# Autodesk Inventor assembly: 4x1inTractionWheel(Tire)-1111-2016_MIR
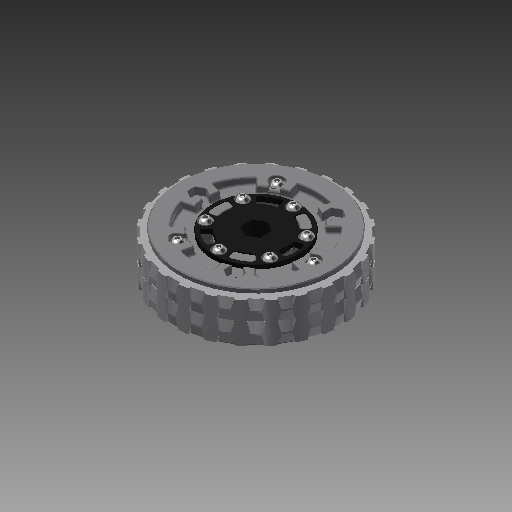
[picture p0: Inventor's stored thumbnail of the model, 512x512]
Saved by Autodesk Inventor 2018 (Build 220112000, 112)
## iProperties
Created: 2016-11-21
Part Number: 4x1inTractionWheel(Tire)-1111-2016_MIR
Document SubType Name: Assembly
Designer: Power Hawks CADD
Mass: 261.422 g
Surface Area: 1262.82 cm^2
Volume: 193.241 cm^3
Density: 1.35283 g/cm^3
Author: 589013
## Documents named in this file (9)
- F:\GrabCad\Resources\VEXpro Resources\Wheels\4 inch\4x1inTractionWheel(Tire)-1111-2016_MIR.iam
- F:\GrabCad\Resources\VEXpro Resources\Wheels\Wheel Parts\4InchWheelEnd-1111-2016_MIR.ipt
- F:\GrabCad\Resources\VEXpro Resources\Fasteners\Standoffs\Standoff0.75in-1111-2016_MIR.ipt
- F:\GrabCad\Resources\VEXpro Resources\Fasteners\Screws\Screw8-32x1.25in-1111-2016_MIR.ipt
- F:\GrabCad\Resources\VEXpro Resources\Fasteners\Nuts\Nut8-32Nylock-1111-2016_MIR.ipt
- F:\GrabCad\Resources\VEXpro Resources\Versa Motion\VersaHub(0.5inHex)-1111-2016_MIR.ipt
- F:\GrabCad\Resources\VEXpro Resources\Versa Motion\VersaHub(0.5inHex,Plastic)-1111-2016_MIR.ipt
- F:\GrabCad\Resources\VEXpro Resources\Fasteners\Screws\Screw8-32x0.5in-1111-2016_MIR.ipt
- F:\GrabCad\Resources\VEXpro Resources\Wheels\Wheel Parts\4InchTire\4inchTire-1111-2017_MIR.iam
## Components (30 placed, 8 different names)
1. 4InchWheelEnd-1111-2016_MIR:1 — Angle:1, Angle:2, Angle:4, Angle:3, Rotational:1, Rotational:3, Rotational:2, Rotational:6, Rotational:5, Rotational:4, Rotational:10, Rotational:9, Rigid:1
2. 4InchWheelEnd-1111-2016_MIR:2 — Insert:1, Insert:2, Insert:3, Rotational:3, Rotational:2, Rotational:8, Rotational:7, Rigid:2
3. Screw8-32x1.25in-1111-2016_MIR:1 — Insert:1
4. Screw8-32x1.25in-1111-2016_MIR:2 — Insert:2
5. Screw8-32x1.25in-1111-2016_MIR:3 — Insert:3
6. Nut8-32Nylock-1111-2016_MIR:1 — Angle:2, Rotational:6
7. Nut8-32Nylock-1111-2016_MIR:2 — Angle:4, Rotational:5
8. Nut8-32Nylock-1111-2016_MIR:3 — Angle:3, Rotational:4
9. VersaHub(0.5inHex)-1111-2016_MIR:1 — Insert:4, Insert:6, Insert:5, Insert:7, Insert:8, Insert:9, Rotational:8, Rotational:7
10. VersaHub(0.5inHex,Plastic)-1111-2016_MIR:1 — Insert:10, Insert:11, Insert:13, Insert:14, Insert:12, Insert:15, Rotational:10, Rotational:9
11. Screw8-32x0.5in-1111-2016_MIR:1 — Insert:4
12. Screw8-32x0.5in-1111-2016_MIR:2 — Insert:6
13. Screw8-32x0.5in-1111-2016_MIR:3 — Insert:5
14. Screw8-32x0.5in-1111-2016_MIR:4 — Insert:7
15. Screw8-32x0.5in-1111-2016_MIR:5 — Insert:8
16. Screw8-32x0.5in-1111-2016_MIR:6 — Insert:9
17. Screw8-32x0.5in-1111-2016_MIR:7 — Insert:10
18. Screw8-32x0.5in-1111-2016_MIR:8 — Insert:11
19. Screw8-32x0.5in-1111-2016_MIR:9 — Insert:13
20. Screw8-32x0.5in-1111-2016_MIR:10 — Insert:14
21. Screw8-32x0.5in-1111-2016_MIR:11 — Insert:12
22. Screw8-32x0.5in-1111-2016_MIR:12 — Insert:15
23. 4inchTire-1111-2017_MIR:1 [sub-assembly] — Rigid:1
24. 4inchTire-1111-2017_MIR:2 [sub-assembly] — Rigid:2
25. Standoff0.75in-1111-2016_MIR:1 — Angle:1, Rotational:1
26. Standoff0.75in-1111-2016_MIR:2
27. Standoff0.75in-1111-2016_MIR:3
28. Standoff0.75in-1111-2016_MIR:4
29. Standoff0.75in-1111-2016_MIR:5
30. Standoff0.75in-1111-2016_MIR:6
## Component patterns: (6 elements, first: Standoff0.75in-1111-2016_MIR:1)
## Relationships (31: Insert 15, RevoluteJoint 10, Angle 4, WeldJoint 2)
- Angle:1 (0 deg): 4InchWheelEnd-1111-2016_MIR:1 ↔ Standoff0.75in-1111-2016_MIR:1
- Insert:1: 4InchWheelEnd-1111-2016_MIR:2 ↔ Screw8-32x1.25in-1111-2016_MIR:1
- Insert:2: 4InchWheelEnd-1111-2016_MIR:2 ↔ Screw8-32x1.25in-1111-2016_MIR:2
- Insert:3: 4InchWheelEnd-1111-2016_MIR:2 ↔ Screw8-32x1.25in-1111-2016_MIR:3
- Angle:2 (0 deg): 4InchWheelEnd-1111-2016_MIR:1 ↔ Nut8-32Nylock-1111-2016_MIR:1
- Angle:4 (0 deg): 4InchWheelEnd-1111-2016_MIR:1 ↔ Nut8-32Nylock-1111-2016_MIR:2
- Angle:3 (0 deg): 4InchWheelEnd-1111-2016_MIR:1 ↔ Nut8-32Nylock-1111-2016_MIR:3
- Insert:4: VersaHub(0.5inHex)-1111-2016_MIR:1 ↔ Screw8-32x0.5in-1111-2016_MIR:1
- Insert:6: VersaHub(0.5inHex)-1111-2016_MIR:1 ↔ Screw8-32x0.5in-1111-2016_MIR:2
- Insert:5: VersaHub(0.5inHex)-1111-2016_MIR:1 ↔ Screw8-32x0.5in-1111-2016_MIR:3
- Insert:7: VersaHub(0.5inHex)-1111-2016_MIR:1 ↔ Screw8-32x0.5in-1111-2016_MIR:4
- Insert:8: VersaHub(0.5inHex)-1111-2016_MIR:1 ↔ Screw8-32x0.5in-1111-2016_MIR:5
- Insert:9: VersaHub(0.5inHex)-1111-2016_MIR:1 ↔ Screw8-32x0.5in-1111-2016_MIR:6
- Insert:10: VersaHub(0.5inHex,Plastic)-1111-2016_MIR:1 ↔ Screw8-32x0.5in-1111-2016_MIR:7
- Insert:11: VersaHub(0.5inHex,Plastic)-1111-2016_MIR:1 ↔ Screw8-32x0.5in-1111-2016_MIR:8
- Insert:13: VersaHub(0.5inHex,Plastic)-1111-2016_MIR:1 ↔ Screw8-32x0.5in-1111-2016_MIR:9
- Insert:14: VersaHub(0.5inHex,Plastic)-1111-2016_MIR:1 ↔ Screw8-32x0.5in-1111-2016_MIR:10
- Insert:12: VersaHub(0.5inHex,Plastic)-1111-2016_MIR:1 ↔ Screw8-32x0.5in-1111-2016_MIR:11
- Insert:15: VersaHub(0.5inHex,Plastic)-1111-2016_MIR:1 ↔ Screw8-32x0.5in-1111-2016_MIR:12
- Rotational:1 [RevoluteJoint]: 4InchWheelEnd-1111-2016_MIR:1 ↔ Standoff0.75in-1111-2016_MIR:1
- Rotational:3 [RevoluteJoint]: 4InchWheelEnd-1111-2016_MIR:1 ↔ 4InchWheelEnd-1111-2016_MIR:2
- Rotational:2 [RevoluteJoint]: 4InchWheelEnd-1111-2016_MIR:1 ↔ 4InchWheelEnd-1111-2016_MIR:2
- Rotational:6 [RevoluteJoint]: 4InchWheelEnd-1111-2016_MIR:1 ↔ Nut8-32Nylock-1111-2016_MIR:1
- Rotational:5 [RevoluteJoint]: 4InchWheelEnd-1111-2016_MIR:1 ↔ Nut8-32Nylock-1111-2016_MIR:2
- Rotational:4 [RevoluteJoint]: 4InchWheelEnd-1111-2016_MIR:1 ↔ Nut8-32Nylock-1111-2016_MIR:3
- Rotational:8 [RevoluteJoint]: 4InchWheelEnd-1111-2016_MIR:2 ↔ VersaHub(0.5inHex)-1111-2016_MIR:1
- Rotational:7 [RevoluteJoint]: 4InchWheelEnd-1111-2016_MIR:2 ↔ VersaHub(0.5inHex)-1111-2016_MIR:1
- Rotational:10 [RevoluteJoint]: 4InchWheelEnd-1111-2016_MIR:1 ↔ VersaHub(0.5inHex,Plastic)-1111-2016_MIR:1
- Rotational:9 [RevoluteJoint]: 4InchWheelEnd-1111-2016_MIR:1 ↔ VersaHub(0.5inHex,Plastic)-1111-2016_MIR:1
- Rigid:1 [WeldJoint]: 4InchWheelEnd-1111-2016_MIR:1 ↔ 4inchTire-1111-2017_MIR:1
- Rigid:2 [WeldJoint]: 4InchWheelEnd-1111-2016_MIR:2 ↔ 4inchTire-1111-2017_MIR:2
